# Autodesk Inventor assembly: Link3
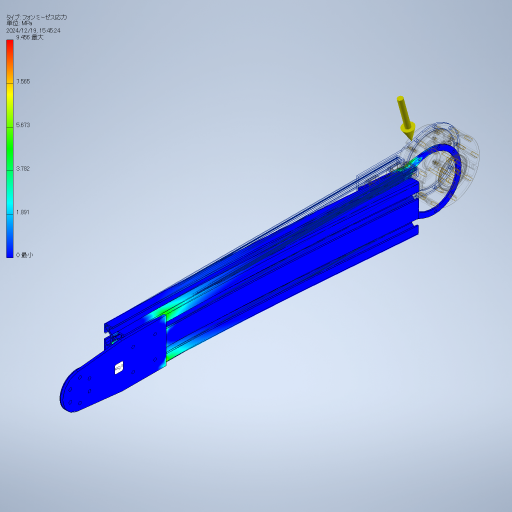
[picture p0: Inventor's stored thumbnail of the model, 512x512]
Saved by Autodesk Inventor 2024 (Build 280153000, 153)
## iProperties
Created: 2024-12-13
Part Number: Link3
Document SubType Name: Assembly
Designer: hirek
Author: hirek
## Documents named in this file (13)
- E:\Documents\Inventor\CanAloha\Link3.iam
- E:\Documents\Inventor\CanAloha\official\robStride02\robStride02.iam
- E:\Documents\Inventor\CanAloha\official\NFSL6-3060\NFSL6-3060-700.ipt
- E:\Documents\Inventor\CanAloha\myperts\link2_plate5.ipt
- E:\Documents\Inventor\CanAloha\myperts\link3_plate1.ipt
- E:\Documents\Inventor\CanAloha\official\HNTT6-4\AIS2024\HNTT6-4.ipt
- E:\Documents\Inventor\CanAloha\myperts\link3_plate2.ipt
- E:\Documents\Inventor\CanAloha\Link3\AIP\FEA\ex0xb8rz4.fins
- E:\Documents\Inventor\CanAloha\Link3\AIP\FEA\ex0xb8s0w.fsat
- E:\Documents\Inventor\CanAloha\Link3\AIP\FEA\ex0xb8s0w.ftes
- E:\Documents\Inventor\CanAloha\Link3\AIP\FEA\ex0xb8s0w.fwiz
- E:\Documents\Inventor\CanAloha\Link3\AIP\FEA\ex0xb8s0x.fmsh
- E:\Documents\Inventor\CanAloha\Link3\AIP\FEA\ex0xb8s0y.fres
## Components (13 placed, 6 different names)
1. NFSL6-3060-700:1 — メイト:1, メイト:2, メイト:3, メイト:4, メイト:5, メイト:6, メイト:7, メイト:8, フラッシュ:1, メイト:9, メイト:10, メイト:11, メイト:12, メイト:13, メイト:14, メイト:15, メイト:16, フラッシュ:2
2. robStride02:1 [sub-assembly] — 回転:7, 回転:12
3. link2_plate5:1 — 回転:5, 回転:6
4. link3_plate1:1 — 回転:1, 回転:2, 回転:3, 回転:4, 回転:5, 回転:6
5. HNTT6-4:1 — メイト:2, メイト:7, 回転:2
6. HNTT6-4:3 — メイト:1, メイト:5, 回転:1
7. HNTT6-4:4 — メイト:3, メイト:6, 回転:3, フラッシュ:1
8. HNTT6-4:5 — メイト:4, メイト:8, 回転:4
9. link3_plate2:1 — 回転:7, 回転:12, 回転:13, 回転:14, 回転:15, 回転:16
10. HNTT6-4:6 — メイト:9, メイト:13, 回転:13
11. HNTT6-4:7 — メイト:10, メイト:14, 回転:15, フラッシュ:2
12. HNTT6-4:8 — メイト:11, メイト:15, 回転:14
13. HNTT6-4:9 — メイト:12, メイト:16, 回転:16
## Relationships (30: Mate 16, RevoluteJoint 12, Flush 2)
- メイト:1 [Mate]: NFSL6-3060-700:1 ↔ HNTT6-4:3
- メイト:2 [Mate]: NFSL6-3060-700:1 ↔ HNTT6-4:1
- メイト:3 [Mate]: NFSL6-3060-700:1 ↔ HNTT6-4:4
- メイト:4 [Mate]: NFSL6-3060-700:1 ↔ HNTT6-4:5
- メイト:5 [Mate]: NFSL6-3060-700:1 ↔ HNTT6-4:3
- メイト:6 [Mate]: NFSL6-3060-700:1 ↔ HNTT6-4:4
- メイト:7 [Mate]: NFSL6-3060-700:1 ↔ HNTT6-4:1
- メイト:8 [Mate]: NFSL6-3060-700:1 ↔ HNTT6-4:5
- 回転:1 [RevoluteJoint] (-1.2 mm): link3_plate1:1 ↔ HNTT6-4:3
- 回転:2 [RevoluteJoint] (-1.2 mm): link3_plate1:1 ↔ HNTT6-4:1
- 回転:3 [RevoluteJoint] (-1.2 mm): link3_plate1:1 ↔ HNTT6-4:4
- 回転:4 [RevoluteJoint] (-1.2 mm): link3_plate1:1 ↔ HNTT6-4:5
- フラッシュ:1 [Flush]: NFSL6-3060-700:1 ↔ HNTT6-4:4
- 回転:5 [RevoluteJoint]: link2_plate5:1 ↔ link3_plate1:1
- 回転:6 [RevoluteJoint]: link2_plate5:1 ↔ link3_plate1:1
- メイト:9 [Mate]: NFSL6-3060-700:1 ↔ HNTT6-4:6
- メイト:10 [Mate]: NFSL6-3060-700:1 ↔ HNTT6-4:7
- メイト:11 [Mate]: NFSL6-3060-700:1 ↔ HNTT6-4:8
- メイト:12 [Mate]: NFSL6-3060-700:1 ↔ HNTT6-4:9
- メイト:13 [Mate]: NFSL6-3060-700:1 ↔ HNTT6-4:6
- メイト:14 [Mate]: NFSL6-3060-700:1 ↔ HNTT6-4:7
- メイト:15 [Mate]: NFSL6-3060-700:1 ↔ HNTT6-4:8
- メイト:16 [Mate]: NFSL6-3060-700:1 ↔ HNTT6-4:9
- 回転:7 [RevoluteJoint]: robStride02:1 ↔ link3_plate2:1
- 回転:12 [RevoluteJoint]: robStride02:1 ↔ link3_plate2:1
- 回転:13 [RevoluteJoint] (-1.2 mm): link3_plate2:1 ↔ HNTT6-4:6
- 回転:14 [RevoluteJoint] (-1.2 mm): link3_plate2:1 ↔ HNTT6-4:8
- 回転:15 [RevoluteJoint] (-1.2 mm): link3_plate2:1 ↔ HNTT6-4:7
- 回転:16 [RevoluteJoint] (-1.2 mm): link3_plate2:1 ↔ HNTT6-4:9
- フラッシュ:2 [Flush]: NFSL6-3060-700:1 ↔ HNTT6-4:7
## Named parameters: sa_0 = 5000
note: some values were not read from the file. Shown as the stored number, unit unknown: "sa_0".
